# Autodesk Inventor assembly: Full assembly
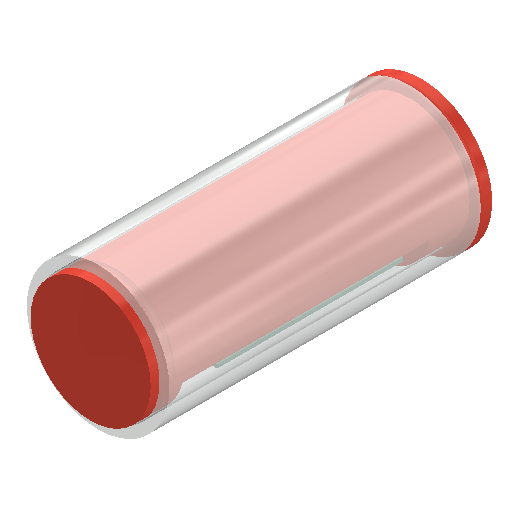
[picture p0: Inventor's stored thumbnail of the model, 512x512]
Saved by Autodesk Inventor 2025 (Build 290162000, 162)
## iProperties
Created: 2025-04-16
Part Number: Full assembly
Document SubType Name: Assembly
Designer: AdminForWorker
Title: Full assembly v12
Author: AdminForWorker
## Documents named in this file (5)
- C:\Users\MK92\OneDrive - University of South Carolina\UAV-Deployable-Stage-Height-Sensor\system_design\Georgetown\V0.5\CAD\Full assembly - Inventor files\Full assembly.iam
- C:\Users\MK92\OneDrive - University of South Carolina\UAV-Deployable-Stage-Height-Sensor\system_design\Georgetown\V0.5\CAD\Full assembly - Inventor files\PCB tray CAD v2.ipt
- C:\Users\MK92\OneDrive - University of South Carolina\UAV-Deployable-Stage-Height-Sensor\system_design\Georgetown\V0.5\CAD\Full assembly - Inventor files\Clear Tube v19.iam
- C:\Users\MK92\OneDrive - University of South Carolina\UAV-Deployable-Stage-Height-Sensor\system_design\Georgetown\V0.5\CAD\Full assembly - Inventor files\main_board v1.iam
- C:\Users\MK92\OneDrive - University of South Carolina\UAV-Deployable-Stage-Height-Sensor\system_design\Georgetown\V0.5\CAD\Full assembly - Inventor files\Battery.ipt
## Components (4 placed, 4 different names)
1. PCB tray CAD v2:1 — Rotation/Translation:1
2. Clear Tube v19:1 [sub-assembly] — Rotation/Translation:1
3. main_board v1:1 [sub-assembly]
4. Battery:1
## Relationships (1: RelateRotateTranslate 1)
- Rotation/Translation:1 [RelateRotateTranslate] (159.517 mm): PCB tray CAD v2:1 ↔ Clear Tube v19:1
